# Autodesk Inventor assembly: Surub M4 saiba piulita
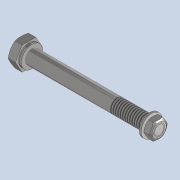
[picture p0: Inventor's stored thumbnail of the model, 180x180]
Saved by Autodesk Inventor 2020 (Build 240168000, 168)
## iProperties
Created: 2020-12-19
Part Number: Surub M4 saiba piulita
Document SubType Name: Assembly
Designer: Iulian Bors
Author: Iulian Bors
## Documents named in this file (4)
- Z:\I.A.B\Proiecte\0005 I.A.B 3d 2.0 Imprimanta aracet\10 Mecanic\Surub M4 saiba piulita.iam
- Z:\I.A.B\Proiecte\0005 I.A.B 3d 2.0 Imprimanta aracet\10 Mecanic\0005-10-1013 ISO 7089 - 4 - 140 HV.ipt
- Z:\I.A.B\Proiecte\0005 I.A.B 3d 2.0 Imprimanta aracet\10 Mecanic\0005-10-1014 ISO 4032 - M4 - ISO.ipt
- C:\Users\40743\Documents\Inventor\Content Center Files\R2020\en-US\ISO 4017(1)\ISO 4017 - M4 x 40 - ISO.ipt
## Components (4 placed, 3 different names)
1. ISO 4017 M4 x 40:1
2. ISO 7089 4:1
3. ISO 4032 M4:1 — Insert:1
4. ISO 7089 4:2 — Insert:1
## Relationships (4: Mate 2, Insert 2)
- [Mate]: ISO 4017 M4 x 40:1 ↔ ISO 7089 4:1
- [Mate]: ISO 4017 M4 x 40:1 ↔ ISO 7089 4:1
- Insert:1: ISO 4032 M4:1 ↔ ISO 7089 4:2
- [Insert]: ISO 4017 M4 x 40:1 ↔ ISO 4032 M4:1
